# Autodesk Inventor assembly: FlyWheelAssembly2
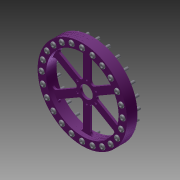
[picture p0: Inventor's stored thumbnail of the model, 180x180]
Saved by Autodesk Inventor 2012 (Build 160160000, 160)
## iProperties
Created: 2012-01-22
Part Number: FlyWheelAssembly2
Document SubType Name: Assembly
Designer: Logan
Author: Logan
## Documents named in this file (4)
- C:\Users\Logan\Desktop\FRC CAD Files\FlyWheelAssembly2.iam
- C:\Users\Logan\Desktop\team1885frc\Robot2012\Shooter\FlyWheelBase.ipt
- C:\Users\Logan\Desktop\team1885frc\Robot2012\Shooter\FlyWheelWeight.ipt
- C:\Users\Logan\Desktop\team1885frc\Robot2012\Shooter\ShooterWeight.ipt
## Components (29 placed, 3 different names)
1. FlyWheelBase:1 — Mate:8, Mate:9, Mate:10, Mate:11
2. FlyWheelWeight:1 — Mate:1, Mate:7, Mate:8, Mate:9
3. FlyWheelWeight:2 — Mate:1, Mate:7, Mate:14, Tangent:1
4. FlyWheelWeight:3 — Mate:10, Mate:11, Mate:12, Mate:13
5. FlyWheelWeight:4 — Mate:12, Mate:13
6. ShooterWeight:1 — Mate:14, Tangent:1
7. ShooterWeight:2
8. ShooterWeight:3
9. ShooterWeight:4
10. ShooterWeight:5
11. ShooterWeight:6
12. ShooterWeight:7
13. ShooterWeight:8
14. ShooterWeight:9
15. ShooterWeight:10
16. ShooterWeight:11
17. ShooterWeight:12
18. ShooterWeight:13
19. ShooterWeight:14
20. ShooterWeight:15
21. ShooterWeight:16
22. ShooterWeight:17
23. ShooterWeight:18
24. ShooterWeight:19
25. ShooterWeight:20
26. ShooterWeight:21
27. ShooterWeight:22
28. ShooterWeight:23
29. ShooterWeight:24
## Component patterns: (24 elements, first: ShooterWeight:1)
## Relationships (10: Mate 9, Tangent 1)
- Mate:1: FlyWheelWeight:1 ↔ FlyWheelWeight:2
- Mate:7: FlyWheelWeight:1 ↔ FlyWheelWeight:2
- Mate:8: FlyWheelBase:1 ↔ FlyWheelWeight:1
- Mate:9: FlyWheelBase:1 ↔ FlyWheelWeight:1
- Mate:10: FlyWheelBase:1 ↔ FlyWheelWeight:3
- Mate:11: FlyWheelBase:1 ↔ FlyWheelWeight:3
- Mate:12: FlyWheelWeight:3 ↔ FlyWheelWeight:4
- Mate:13: FlyWheelWeight:3 ↔ FlyWheelWeight:4
- Mate:14: FlyWheelWeight:2 ↔ ShooterWeight:1
- Tangent:1: FlyWheelWeight:2 ↔ ShooterWeight:1
